# Autodesk Inventor assembly: SPE27V1 Soporte Freno
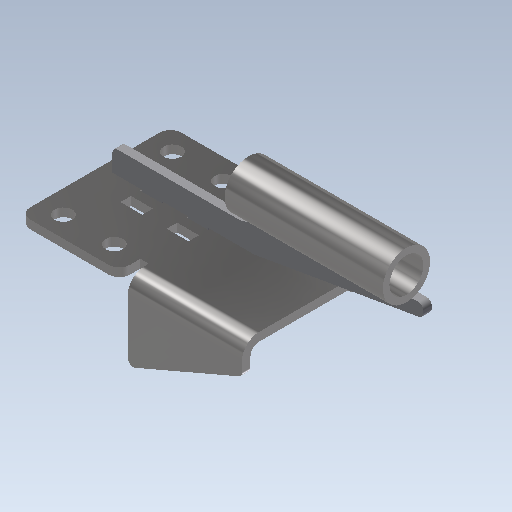
[picture p0: Inventor's stored thumbnail of the model, 512x512]
Saved by Autodesk Inventor 2021.2 (Build 252289000, 289)
## iProperties
Created: 2026-08-04
Part Number: SPE27V1 Soporte Freno
Document SubType Name: Assembly
Designer: nelso
Author: nelso
## Documents named in this file (4)
- C:\Users\nelso\Desktop\Soporte-Paciente-Espinografia\Workspace\SPE27V1 Soporte Freno.iam
- C:\Users\nelso\Desktop\Soporte-Paciente-Espinografia\Workspace\SP10V1 Estructura Freno.ipt
- C:\Users\nelso\Desktop\Soporte-Paciente-Espinografia\Workspace\SP9V1 Columna Freno.ipt
- C:\Users\nelso\Desktop\Soporte-Paciente-Espinografia\Workspace\SP5V1 Camisa Freno.ipt
## Components (3 placed, 3 different names)
1. SP10V1 Estructura Freno:1
2. SP9V1 Columna Freno:1
3. SP5V1 Camisa Freno:1
## Relationships (3: Mate 2, Flush 1)
- [Mate]: SP10V1 Estructura Freno:1 ↔ SP9V1 Columna Freno:1
- [Mate]: SP10V1 Estructura Freno:1 ↔ SP9V1 Columna Freno:1
- [Flush]: SP9V1 Columna Freno:1 ↔ SP5V1 Camisa Freno:1
